# Autodesk Inventor assembly: Koppeltest_Aufhängung
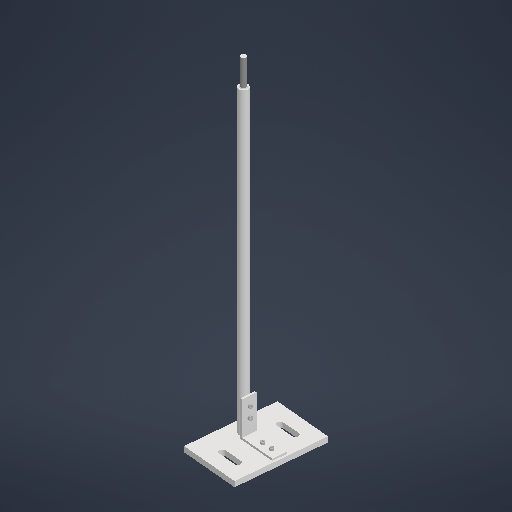
[picture p0: Inventor's stored thumbnail of the model, 512x512]
Saved by Autodesk Inventor 2027 (Build 310192060, 192F)
## iProperties
Created: 2026-06-23
Part Number: Koppeltest_Aufhängung
Document SubType Name: Assembly
Designer: kw
Author: kw
## Documents named in this file (7)
- C:\Users\kw\OneDrive\Documents\Uni\Masterthesis\Spezialisierungsmodul\InventorZeichnungen\Koppeltest_Halterung\Koppeltest_Halterung.iam
- C:\Users\kw\OneDrive\Documents\Uni\Masterthesis\Spezialisierungsmodul\InventorZeichnungen\Koppeltest_Halterung\Halterung_Führungsschiene.ipt
- C:\Users\kw\OneDrive\Documents\Uni\Masterthesis\Spezialisierungsmodul\InventorZeichnungen\Koppeltest_Halterung\Halterung_Stange.ipt
- C:\Users\kw\OneDrive\Documents\Uni\Masterthesis\Spezialisierungsmodul\InventorZeichnungen\M6X20_Countersunk.ipt
- C:\Users\kw\OneDrive\Documents\Uni\Masterthesis\Spezialisierungsmodul\InventorZeichnungen\Koppeltest_Halterung\Winkel_Stange.ipt
- C:\Users\kw\OneDrive\Documents\Uni\Masterthesis\Spezialisierungsmodul\InventorZeichnungen\M3X10_SHCS.ipt
- C:\Users\kw\OneDrive\Documents\Uni\Masterthesis\Spezialisierungsmodul\InventorZeichnungen\M3X16_SHCS.ipt
## Components (8 placed, 6 different names)
1. Halterung_Führungsschiene:1 — Mate:16, Flush:5, Mate:17, Mate:18, Mate:19, Flush:6
2. M6X20_Countersunk:1 — Mate:16, Flush:5
3. Halterung_Stange:1 — Mate:17, Mate:18, Mate:20, Mate:21, Mate:22
4. Winkel_Stange:1 — Mate:19, Mate:20, Mate:21, Mate:22, Flush:6, Mate:23, Mate:24, Mate:25, Mate:26, Mate:27, Mate:28, Mate:29, Mate:30
5. M3X10_SHCS:1 — Mate:23, Mate:25
6. M3X16_SHCS:1 — Mate:27, Mate:29
7. M3X10_SHCS:2 — Mate:24, Mate:26
8. M3X16_SHCS:2 — Mate:28, Mate:30
## Relationships (17: Mate 15, Flush 2)
- Mate:16: Halterung_Führungsschiene:1 ↔ M6X20_Countersunk:1
- Flush:5: Halterung_Führungsschiene:1 ↔ M6X20_Countersunk:1
- Mate:17: Halterung_Führungsschiene:1 ↔ Halterung_Stange:1
- Mate:18: Halterung_Führungsschiene:1 ↔ Halterung_Stange:1
- Mate:19: Halterung_Führungsschiene:1 ↔ Winkel_Stange:1
- Mate:20 (7 mm): Halterung_Stange:1 ↔ Winkel_Stange:1
- Mate:21: Halterung_Stange:1 ↔ Winkel_Stange:1
- Mate:22: Halterung_Stange:1 ↔ Winkel_Stange:1
- Flush:6 (3 mm): Halterung_Führungsschiene:1 ↔ Winkel_Stange:1
- Mate:23: Winkel_Stange:1 ↔ M3X10_SHCS:1
- Mate:24: Winkel_Stange:1 ↔ M3X10_SHCS:2
- Mate:25: Winkel_Stange:1 ↔ M3X10_SHCS:1
- Mate:26: Winkel_Stange:1 ↔ M3X10_SHCS:2
- Mate:27: Winkel_Stange:1 ↔ M3X16_SHCS:1
- Mate:28: Winkel_Stange:1 ↔ M3X16_SHCS:2
- Mate:29: Winkel_Stange:1 ↔ M3X16_SHCS:1
- Mate:30: Winkel_Stange:1 ↔ M3X16_SHCS:2
